# Autodesk Inventor assembly: Sideways pulley mount 2
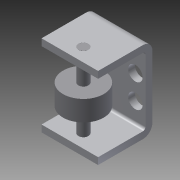
[picture p0: Inventor's stored thumbnail of the model, 180x180]
Saved by Autodesk Inventor 2013 (Build 170138000, 138)
## iProperties
Created: 2013-02-07
Part Number: Sideways pulley mount 2
Document SubType Name: Assembly
Designer: Arpan
Mass: 20.5392 g
Surface Area: 67.8393 cm^2
Volume: 9.61328 cm^3
Density: 2.13654 g/cm^3
Author: Arpan
## Documents named in this file (4)
- C:\Users\Moses\Documents\GitHub\frc2013CAD\M-Climber\Sideways pulley mount 2.iam
- C:\Users\Moses\Documents\GitHub\frc2013CAD\M-Climber\3 16ths shaft.ipt
- C:\Users\Moses\Documents\GitHub\frc2013CAD\M-Climber\1 8th pulley.ipt
- C:\Users\Moses\Documents\GitHub\frc2013CAD\M-Climber\pulley mount actual sideways left.ipt
## Components (3 placed, 3 different names)
1. 3 16ths shaft:1 — Mate:2, Mate:3, Flush:1
2. 1 8th pulley:1 — Mate:2, Mate:4
3. pulley mount actual sideways left:1 — Mate:3, Flush:1, Mate:4
## Relationships (4: Mate 3, Flush 1)
- Mate:2: 3 16ths shaft:1 ↔ 1 8th pulley:1
- Mate:3: 3 16ths shaft:1 ↔ pulley mount actual sideways left:1
- Flush:1: 3 16ths shaft:1 ↔ pulley mount actual sideways left:1
- Mate:4 (11.2268 mm): 1 8th pulley:1 ↔ pulley mount actual sideways left:1
